# Autodesk Inventor assembly: pedestal assembly
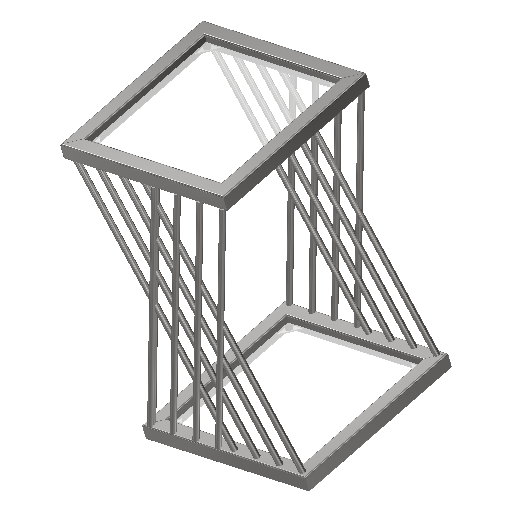
[picture p0: Inventor's stored thumbnail of the model, 512x512]
Saved by Autodesk Inventor 2025 (Build 290162000, 162)
## iProperties
Created: 2024-09-24
Part Number: pedestal assembly
Document SubType Name: Assembly
Designer: teiko
Author: teiko
## Documents named in this file (6)
- C:\Users\teiko\OneDrive\Documents\Inventor\pedestal table\assembly\pedestal assembly.iam
- C:\Users\teiko\OneDrive\Documents\Inventor\pedestal table\parts\Assembly1.iam
- C:\Users\teiko\OneDrive\Documents\Inventor\pedestal table\parts\internal member.ipt
- C:\Users\teiko\OneDrive\Documents\Inventor\pedestal table\parts\internal member_MIR.ipt
- C:\Users\teiko\OneDrive\Documents\Inventor\pedestal table\parts\round piece.ipt
- C:\Users\teiko\OneDrive\Documents\Inventor\pedestal table\parts\pedestal glass.ipt
## Components (33 placed, 5 different names)
1. Assembly1:1 [sub-assembly] — Mate:1, Flush:1, Flush:2, Mate:4, Mate:5, Mate:6, Flush:4, Mate:7, Mate:8, Mate:9, Mate:10, Mate:11, Mate:12, Mate:13, Mate:14, Mate:16, Mate:17
2. Assembly1:2 [sub-assembly] — Mate:1, Flush:1, Flush:2, Mate:2, Flush:3, Mate:3
3. internal member:13 — Mate:7, Mate:8
4. internal member_MIR:1
5. internal member_MIR:2
6. internal member_MIR:3
7. internal member_MIR:4
8. internal member_MIR:5
9. internal member_MIR:6
10. internal member_MIR:7
11. internal member_MIR:8
12. internal member:1 — Mate:2, Flush:3, Mate:3, Flush:5
13. internal member:2
14. internal member:3
15. internal member:4
16. internal member:5 — Mate:4, Mate:5
17. internal member:6
18. internal member:7
19. internal member:8
20. internal member:9 — Mate:6, Flush:4
21. internal member:10
22. internal member:11
23. internal member:12
24. pedestal glass:1 — Mate:15, Mate:16, Mate:17
25. pedestal glass:2
26. round piece:1 — Mate:9, Mate:10, Mate:11, Mate:15
27. round piece:2 — Mate:12, Mate:13, Mate:14
28. round piece:3
29. round piece:4
30. round piece:5
31. round piece:6
32. round piece:7
33. round piece:8
## Component patterns: (4 elements, first: internal member:1), (4 elements, first: internal member:5), (4 elements, first: internal member:9), (2 elements, first: pedestal glass:1), (2 elements, first: round piece:1 + round piece:2), Component Pattern 5:2 (2 elements)
## Relationships (22: Mate 17, Flush 5)
- Mate:1 (450 mm): Assembly1:1 ↔ Assembly1:2
- Flush:1: Assembly1:1 ↔ Assembly1:2
- Flush:2: Assembly1:1 ↔ Assembly1:2
- Mate:2: Assembly1:2 ↔ internal member:1
- Flush:3: Assembly1:2 ↔ internal member:1
- Mate:3: Assembly1:2 ↔ internal member:1
- Mate:4: Assembly1:1 ↔ internal member:5
- Mate:5: Assembly1:1 ↔ internal member:5
- Mate:6: Assembly1:1 ↔ internal member:9
- Flush:4: Assembly1:1 ↔ internal member:9
- Flush:5: internal member:1
- Mate:7: Assembly1:1 ↔ internal member:13
- Mate:8: Assembly1:1 ↔ internal member:13
- Mate:9: Assembly1:1 ↔ round piece:1
- Mate:10 (-7 mm): Assembly1:1 ↔ round piece:1
- Mate:11: Assembly1:1 ↔ round piece:1
- Mate:12: Assembly1:1 ↔ round piece:2
- Mate:13 (-7 mm): Assembly1:1 ↔ round piece:2
- Mate:14: Assembly1:1 ↔ round piece:2
- Mate:15: pedestal glass:1 ↔ round piece:1
- Mate:16: Assembly1:1 ↔ pedestal glass:1
- Mate:17: Assembly1:1 ↔ pedestal glass:1
